# Autodesk Inventor assembly: Right Leg
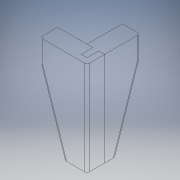
[picture p0: Inventor's stored thumbnail of the model, 180x180]
Saved by Autodesk Inventor 2016 (Build 200138000, 138)
## iProperties
Created: 2017-11-04
Part Number: Right Leg
Document SubType Name: Assembly
Designer: mathaetaes
Author: mathaetaes
## Documents named in this file (3)
- E:\Projects\3D Printer\printer projects\My Designs\Bar Cabinet\Right Leg.iam
- E:\Projects\3D Printer\printer projects\My Designs\Bar Cabinet\Right Leg, Front part.ipt
- E:\Projects\3D Printer\printer projects\My Designs\Bar Cabinet\Right Leg, Side Partt.ipt
## Components (2 placed, 2 different names)
1. Right Leg, Front part:1 — Mate:1, Mate:2, Flush:1
2. Right Leg, Side Partt:1 — Mate:1, Mate:2, Flush:1
## Relationships (3: Mate 2, Flush 1)
- Mate:1: Right Leg, Front part:1 ↔ Right Leg, Side Partt:1
- Mate:2: Right Leg, Front part:1 ↔ Right Leg, Side Partt:1
- Flush:1: Right Leg, Front part:1 ↔ Right Leg, Side Partt:1
